# Autodesk Inventor assembly: IndexL2
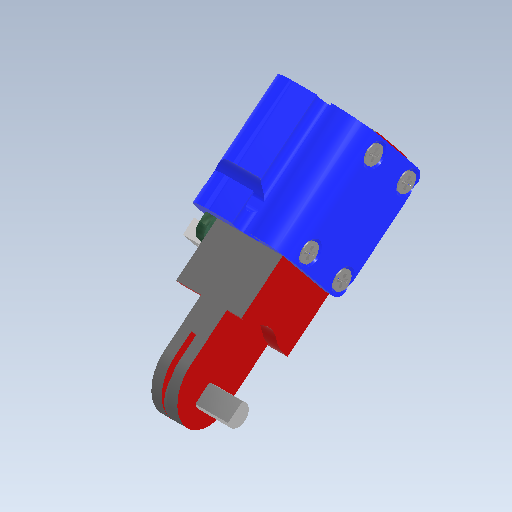
[picture p0: Inventor's stored thumbnail of the model, 512x512]
Saved by Autodesk Inventor 2020 (Build 240168000, 168)
## iProperties
Created: 2020-04-30
Part Number: IndexL2
Document SubType Name: Assembly
Designer: sami_
Author: sami_
## Documents named in this file (10)
- C:\Users\sami_\Documents\V1.6\IndexL2.iam
- C:\Users\sami_\Documents\V1.6\Workgroups\NotInProject\INDEX\L2 Index_MIR.ipt
- C:\Users\sami_\Documents\V1.6\Libraries\Content Center Files\en-US\ISO 1224-1 M\ISO 1224-1 - 17 - 4 x 7 x 2.ipt
- C:\Users\sami_\Documents\V1.6\Libraries\Content Center Files\en-US\ISO 7089\ISO 7089 - 4 - 140 HV(1).ipt
- C:\Users\sami_\Documents\V1.6\Workgroups\NotInProject\INDEX\PotentiometerAssembly.iam
- C:\Users\sami_\Documents\V1.6\Libraries\Content Center Files\en-US\ISO 7089\ISO 7089 - 1.6 - 140 HV(1).ipt
- C:\Users\sami_\Documents\V1.6\Workgroups\NotInProject\fingerpanel.ipt
- C:\Users\sami_\Documents\V1.6\Libraries\Content Center Files\en-US\AS 1427(04)\AS 1427 - M2 x 4(5) I.ipt
- C:\Users\sami_\Documents\V1.6\Libraries\Content Center Files\en-US\AS 1427(04)\AS 1427 - M2 x 8(5) I.ipt
- C:\Users\sami_\Documents\V1.6\Workgroups\NotInProject\SHAFT.ipt
## Components (25 placed, 9 different names)
1. L2 Index_MIR:1
2. ISO 1224-1 (Metric) 17 - 4 x 7 x 2:1
3. SHAFT:1
4. ISO 1224-1 (Metric) 17 - 4 x 7 x 2:2
5. ISO 7089 4:1
6. ISO 7089 4:2
7. PotentiometerAssembly:1 [sub-assembly]
8. ISO 7089 1.6:1
9. ISO 7089 1.6:2
10. ISO 7089 1.6:3
11. ISO 7089 1.6:4
12. fingerpanel:1
13. ISO 7089 1.6:5
14. ISO 7089 1.6:6
15. ISO 7089 1.6:7
16. ISO 7089 1.6:8
17. ISO 7089 1.6:9
18. AS 1427 H - Metric M2 x 4:1
19. AS 1427 H - Metric M2 x 4:2
20. AS 1427 H - Metric M2 x 4:3
21. AS 1427 H - Metric M2 x 4:4
22. AS 1427 H - Metric M2 x 8:1
23. AS 1427 H - Metric M2 x 8:2
24. AS 1427 H - Metric M2 x 8:3
25. AS 1427 H - Metric M2 x 8:4
## Relationships (23: Insert 9, Mate 8, WeldJoint 5, RevoluteJoint 1)
- [WeldJoint] (0.6 mm): L2 Index_MIR:1 ↔ PotentiometerAssembly:1
- [Insert]: L2 Index_MIR:1 ↔ ISO 7089 1.6:1
- [Insert]: L2 Index_MIR:1 ↔ ISO 7089 1.6:2
- [Insert]: L2 Index_MIR:1 ↔ ISO 7089 1.6:3
- [Insert]: L2 Index_MIR:1 ↔ ISO 7089 1.6:4
- [WeldJoint]: ISO 1224-1 (Metric) 17 - 4 x 7 x 2:2 ↔ ISO 7089 4:1
- [WeldJoint]: ISO 1224-1 (Metric) 17 - 4 x 7 x 2:1 ↔ ISO 7089 4:2
- [WeldJoint]: L2 Index_MIR:1 ↔ ISO 7089 4:1
- [RevoluteJoint]: L2 Index_MIR:1 ↔ ISO 7089 4:2
- [Insert]: ISO 7089 1.6:4 ↔ ISO 7089 1.6:5
- [Insert]: PotentiometerAssembly:1 ↔ ISO 7089 1.6:6
- [Insert]: PotentiometerAssembly:1 ↔ ISO 7089 1.6:7
- [Insert]: PotentiometerAssembly:1 ↔ ISO 7089 1.6:8
- [Insert]: PotentiometerAssembly:1 ↔ ISO 7089 1.6:9
- [WeldJoint]: PotentiometerAssembly:1 ↔ fingerpanel:1
- [Mate]: fingerpanel:1 ↔ AS 1427 H - Metric M2 x 4:1
- [Mate]: fingerpanel:1 ↔ AS 1427 H - Metric M2 x 4:2
- [Mate]: fingerpanel:1 ↔ AS 1427 H - Metric M2 x 4:3
- [Mate]: fingerpanel:1 ↔ AS 1427 H - Metric M2 x 4:4
- [Mate]: fingerpanel:1 ↔ AS 1427 H - Metric M2 x 8:1
- [Mate]: fingerpanel:1 ↔ AS 1427 H - Metric M2 x 8:2
- [Mate]: fingerpanel:1 ↔ AS 1427 H - Metric M2 x 8:3
- [Mate]: fingerpanel:1 ↔ AS 1427 H - Metric M2 x 8:4
